# Autodesk Inventor assembly: Propdrive V2 3536D 1400KV
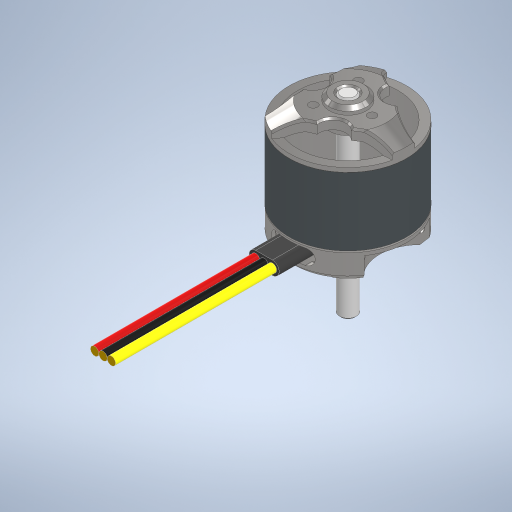
[picture p0: Inventor's stored thumbnail of the model, 512x512]
Saved by Autodesk Inventor 2023.2 (Build 272271000, 271)
## iProperties
Created: 2023-03-04
Part Number: Propdrive V2 3536D 1400KV
Document SubType Name: Assembly
Designer: Nathan Cai
Author: Nathan Cai
## Documents named in this file (5)
- C:\Users\Nathan Cai\Documents\Inventor\Asorted Parts\Propdrive V2 3536D 1400KV\Propdrive V2 3536D 1400KV.iam
- C:\Users\Nathan Cai\Documents\Inventor\Asorted Parts\Propdrive V2 3536D 1400KV\Base.ipt
- C:\Users\Nathan Cai\Documents\Inventor\Asorted Parts\Propdrive V2 3536D 1400KV\Can.ipt
- C:\Users\Nathan Cai\Documents\Inventor\Asorted Parts\Propdrive V2 3536D 1400KV\Cables.ipt
- C:\Users\Nathan Cai\Documents\Inventor\Asorted Parts\Propdrive V2 3536D 1400KV\Shaft.ipt
## Components (4 placed, 4 different names)
1. Base:1 — Mate:1, Mate:2, Mate:3, Flush:1, Mate:4
2. Can:1 — Mate:1, Mate:2, Mate:5, Flush:2
3. Cables:1 — Mate:3, Flush:1, Mate:4
4. Shaft:1 — Mate:5, Flush:2
## Relationships (7: Mate 5, Flush 2)
- Mate:1: Base:1 ↔ Can:1
- Mate:2 (-35 mm): Base:1 ↔ Can:1
- Mate:3: Base:1 ↔ Cables:1
- Flush:1: Base:1 ↔ Cables:1
- Mate:4: Base:1 ↔ Cables:1
- Mate:5: Can:1 ↔ Shaft:1
- Flush:2: Can:1 ↔ Shaft:1
